# Autodesk Inventor assembly: Chain Drive6_MIR
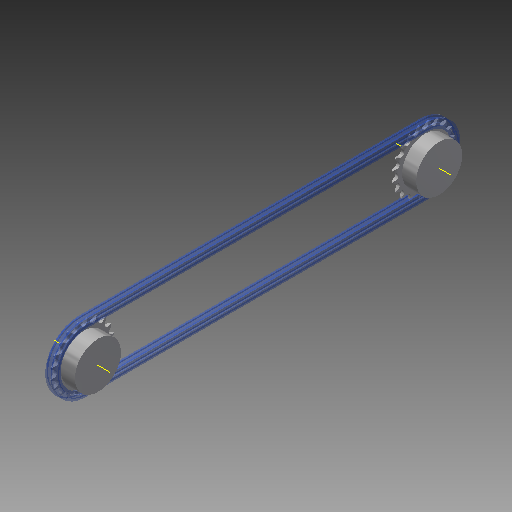
[picture p0: Inventor's stored thumbnail of the model, 512x512]
Saved by Autodesk Inventor 2019.4 (Build 234330000, 330)
## iProperties
Created: 2019-12-08
Part Number: Chain Drive6_MIR
Document SubType Name: Assembly
Designer: admin
Mass: 355.634 g
Surface Area: 387.811 cm^2
Volume: 73.1105 cm^3
Density: 4.86433 g/cm^3
Author: Mark
## Documents named in this file (4)
- C:\Users\admin\Desktop\FRC 2020 Engineering\GitHub\7738-CAD-prep\WCD\WCD V2\Design Accelerator\Chain Drive6_MIR.iam
- C:\Users\admin\Desktop\FRC 2020 Engineering\GitHub\7738-CAD-prep\WCD\WCD V2\Design Accelerator\Roller Chain6_MIR.ipt
- C:\Users\admin\Desktop\FRC 2020 Engineering\GitHub\7738-CAD-prep\WCD\WCD V2\Design Accelerator\Roller Chain Sprocket15_MIR.ipt
- C:\Users\admin\Desktop\FRC 2020 Engineering\GitHub\7738-CAD-prep\WCD\WCD V2\Design Accelerator\Roller Chain Sprocket26_MIR.ipt
## Components (3 placed, 3 different names)
1. Roller Chain6_MIR:1 — Mate:2, Mate:1, Flush:1, Mate:4, Mate:3, Flush:2
2. Roller Chain Sprocket15_MIR:1 — Mate:2, Mate:1, Flush:1, Rotation:1
3. Roller Chain Sprocket26_MIR:1 — Mate:4, Mate:3, Flush:2, Rotation:1
## Relationships (7: Mate 4, Flush 2, RelateRotation 1)
- Mate:2: Roller Chain6_MIR:1 ↔ Roller Chain Sprocket15_MIR:1
- Mate:1: Roller Chain6_MIR:1 ↔ Roller Chain Sprocket15_MIR:1
- Flush:1: Roller Chain6_MIR:1 ↔ Roller Chain Sprocket15_MIR:1
- Mate:4: Roller Chain6_MIR:1 ↔ Roller Chain Sprocket26_MIR:1
- Mate:3: Roller Chain6_MIR:1 ↔ Roller Chain Sprocket26_MIR:1
- Flush:2: Roller Chain6_MIR:1 ↔ Roller Chain Sprocket26_MIR:1
- Rotation:1 [RelateRotation] (1 ul): Roller Chain Sprocket15_MIR:1 ↔ Roller Chain Sprocket26_MIR:1
